# Autodesk Inventor assembly: MainAssy_MIR_MIR
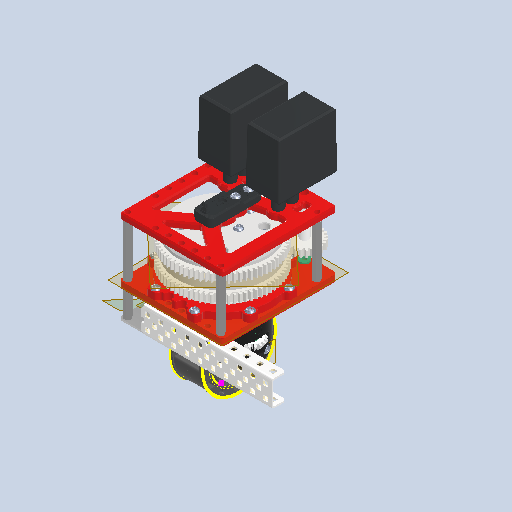
[picture p0: Inventor's stored thumbnail of the model, 512x512]
Saved by Autodesk Inventor 2023 (Build 270158000, 158)
## iProperties
Created: 2022-10-29
Part Number: MainAssy_MIR_MIR
Document SubType Name: Assembly
Designer: zac-h
Author: zac-h
## Documents named in this file (41)
- C:\Users\Zac Hah\Documents\GitHub\spin-up-cad\guardSwerve5\MainAssy_MIR_MIR.iam
- C:\Users\Zac Hah\Documents\GitHub\spin-up-cad\guardSwerve5\WheelHalf_MIR1_MIR.ipt
- C:\Users\Zac Hah\Documents\GitHub\spin-up-cad\guardSwerve5\WheelHalf_MIR_MIR_MIR.ipt
- C:\Users\Zac Hah\Documents\GitHub\spin-up-cad\guardSwerve5\Carriage_MIR_MIR.ipt
- C:\Users\Zac Hah\Documents\GitHub\spin-up-cad\guardSwerve5\MainAssy\Design Accelerator\Bevel Gears1_MIR_MIR.iam
- C:\Users\Zac Hah\Documents\GitHub\spin-up-cad\VEX-CAD-Inventor-1.3.0\VEX-CAD-Inventor-1.3.0\Motion\Circle Insert_MIR_MIR.ipt
- C:\Users\Zac Hah\Documents\GitHub\spin-up-cad\guardSwerve5\Baseplate_MIR_MIR.ipt
- C:\Users\Zac Hah\Documents\GitHub\spin-up-cad\VEX-CAD-Inventor-1.3.0\VEX-CAD-Inventor-1.3.0\Structure\C-Channels\Aluminum 1x2x1\Alu C 1x2x1x10_MIR_MIR.ipt
- C:\Users\Zac Hah\Documents\GitHub\spin-up-cad\guardSwerve5\UpperRaceRing_MIR_MIR.ipt
- C:\Users\Zac Hah\Documents\GitHub\spin-up-cad\guardSwerve5\SteeringCoupler_MIR_MIR.ipt
- C:\Users\Zac Hah\Documents\GitHub\spin-up-cad\guardSwerve5\MainAssy\Design Accelerator\Spur Gears1_MIR_MIR.iam
- C:\Users\Zac Hah\Documents\GitHub\spin-up-cad\guardSwerve5\MainAssy\Design Accelerator\Spur Gears2_MIR_MIR.iam
- C:\Users\Zac Hah\Documents\GitHub\spin-up-cad\guardSwerve5\MainAssy\Design Accelerator\Spur Gears4_MIR_MIR.iam
- C:\Users\Zac Hah\Documents\GitHub\spin-up-cad\guardSwerve5\MainAssy\Design Accelerator\Spur Gears5_MIR_MIR.iam
- C:\Users\Zac Hah\Documents\GitHub\spin-up-cad\guardSwerve5\MainAssy\Design Accelerator\Spur Gears3_MIR_MIR.iam
- C:\Users\Zac Hah\Documents\GitHub\spin-up-cad\guardSwerve5\MainAssy\Design Accelerator\Spur Gears6_MIR_MIR.iam
- C:\Users\Zac Hah\Documents\GitHub\spin-up-cad\guardSwerve5\UpperRingSeat_MIR_MIR.ipt
- C:\Users\Zac Hah\Documents\GitHub\spin-up-cad\VEX-CAD-Inventor-1.3.0\VEX-CAD-Inventor-1.3.0\Structure\Hardware\Screw Steel - Star\SScrew Star Smooth 1.000.ipt
- C:\Users\zac-h\Documents\CAD\VEX-CAD-Inventor-1.3.0\VEX-CAD-Inventor-1.3.0\Structure\Hardware\Screw Steel - Star.ipt
- C:\Users\Zac Hah\Documents\GitHub\spin-up-cad\guardSwerve5\DiffCap_MIR_MIR.ipt
- C:\Users\Zac Hah\Documents\GitHub\spin-up-cad\VEX-CAD-Inventor-1.3.0\VEX-CAD-Inventor-1.3.0\Motion\Square Insert_MIR_MIR.ipt
- C:\Users\Zac Hah\Documents\GitHub\spin-up-cad\VEX-CAD-Inventor-1.3.0\VEX-CAD-Inventor-1.3.0\Structure\Hardware\Screw Steel - Star\SScrew Star Smooth .875.ipt
- C:\Users\Zac Hah\Documents\GitHub\spin-up-cad\VEX-CAD-Inventor-1.3.0\VEX-CAD-Inventor-1.3.0\Structure\Hardware\Nut Nylock_MIR2_MIR.ipt
- C:\Users\Zac Hah\Documents\GitHub\spin-up-cad\VEX-CAD-Inventor-1.3.0\VEX-CAD-Inventor-1.3.0\Motion\Shaft LS\Shaft LS 3.0 in.ipt
- C:\Users\zac-h\Documents\CAD\VEX-CAD-Inventor-1.3.0\VEX-CAD-Inventor-1.3.0\Motion\Shaft LS.ipt
- C:\Users\Zac Hah\Documents\GitHub\spin-up-cad\VEX-CAD-Inventor-1.3.0\VEX-CAD-Inventor-1.3.0\Structure\Hardware\Screw Steel - Star\SScrew Star Smooth 1.750.ipt
- C:\Users\Zac Hah\Documents\GitHub\spin-up-cad\VEX-CAD-Inventor-1.3.0\VEX-CAD-Inventor-1.3.0\Structure\Standoff\Standoff 2.00.ipt
- C:\Users\zac-h\Documents\CAD\VEX-CAD-Inventor-1.3.0\VEX-CAD-Inventor-1.3.0\Structure\Standoff.ipt
- C:\Users\Zac Hah\Documents\GitHub\spin-up-cad\guardSwerve5\TopPlate_MIR_MIR.ipt
- C:\Users\Zac Hah\Documents\GitHub\spin-up-cad\VEX-CAD-Inventor-1.3.0\VEX-CAD-Inventor-1.3.0\Electronics\V5 Simple Motor_MIR2_MIR.ipt
- C:\Users\Zac Hah\Documents\GitHub\spin-up-cad\VEX-CAD-Inventor-1.3.0\VEX-CAD-Inventor-1.3.0\Electronics\Sensors\Potentiometer V2_MIR_MIR.ipt
- C:\Users\Zac Hah\Documents\GitHub\spin-up-cad\VEX-CAD-Inventor-1.3.0\VEX-CAD-Inventor-1.3.0\Structure\Hardware\Screw Steel - Star\SScrew Star Smooth .750.ipt
- C:\Users\Zac Hah\Documents\GitHub\spin-up-cad\VEX-CAD-Inventor-1.3.0\VEX-CAD-Inventor-1.3.0\Structure\Hardware\Screw Steel - Star\SScrew Star Smooth .500.ipt
- C:\Users\Zac Hah\Documents\GitHub\spin-up-cad\guardSwerve5\UnderGusset_MIR_MIR.ipt
- C:\Users\Zac Hah\Documents\GitHub\spin-up-cad\VEX-CAD-Inventor-1.3.0\VEX-CAD-Inventor-1.3.0\Structure\Standoff\Standoff 1.00.ipt
- C:\Users\Zac Hah\Documents\GitHub\spin-up-cad\guardSwerve5\1.2inSpacer_MIR_MIR.ipt
- C:\Users\Zac Hah\Documents\GitHub\spin-up-cad\guardSwerve1\bearingsleeve_MIR2_MIR.ipt
- C:\Users\Zac Hah\Documents\GitHub\spin-up-cad\guardSwerve5\608bearing_MIR_MIR.ipt
- C:\Users\Zac Hah\Documents\GitHub\spin-up-cad\VEX-CAD-Inventor-1.3.0\VEX-CAD-Inventor-1.3.0\Structure\Hardware\Screw Steel - Star\SScrew Star Smooth .250.ipt
- C:\Users\Zac Hah\Documents\GitHub\spin-up-cad\VEX-CAD-Inventor-1.3.0\VEX-CAD-Inventor-1.3.0\Structure\Hardware\Screw Steel - Star\SScrew Star Smooth 1.250.ipt
- C:\Users\Zac Hah\Documents\GitHub\spin-up-cad\VEX-CAD-Inventor-1.3.0\VEX-CAD-Inventor-1.3.0\Motion\0.188 ID x 0.500 OD x 0.196 WD (Radial Bearing) (217-3246).step
## Components (84 placed, 36 different names)
1. WheelHalf_MIR1_MIR:1 — Mate:1
2. WheelHalf_MIR_MIR_MIR:1 — Flush:1, Mate:25, Angle:5
3. Carriage_MIR_MIR:1 — Flush:1, Mate:4, Mate:24, Angle:4, Mate:5, Mate:6, Mate:7, Insert:11, Insert:12, Flush:2, Insert:3, Insert:39, Insert:38, Insert:37, Insert:36
4. Bevel Gears1_MIR_MIR:1 [sub-assembly] — Mate:1, Mate:4, Mate:24, Angle:4, Mate:25, Angle:5
5. Circle Insert_MIR_MIR:1 — Mate:5, Mate:6, Mate:7
6. Circle Insert_MIR_MIR:2 — Insert:49
7. Circle Insert_MIR_MIR:3 — Insert:44
8. Baseplate_MIR_MIR:1 — Flush:2, Insert:14, Insert:21, Insert:15, Insert:16, Flush:3, Flush:4, Insert:28, Insert:27, Insert:69, Insert:66, Insert:67, Insert:68
9. Alu C 1x2x1x10_MIR_MIR:1 — Insert:14, Insert:21, Flush:13, Flush:14
10. Alu C 1x2x1x10_MIR_MIR:2 — Insert:15, Insert:16
11. UpperRaceRing_MIR_MIR:1 — Flush:3, Flush:4, Insert:29
12. SteeringCoupler_MIR_MIR:1 — Flush:5, Insert:31, Mate:20, Mate:21, Insert:32, Insert:33, Insert:34, Flush:8, Insert:45, Insert:63, Insert:64, Insert:65
13. Spur Gears1_MIR_MIR:1 [sub-assembly] — Insert:31, Insert:49, Flush:7
14. Spur Gears2_MIR_MIR:1 [sub-assembly] — Mate:20, Mate:21, Insert:30, Mate:23, Flush:11
15. Spur Gears4_MIR_MIR:1 [sub-assembly] — Insert:30, Mate:23, Flush:11
16. Circle Insert_MIR_MIR:4 — Insert:28, Insert:85
17. Circle Insert_MIR_MIR:5 — Insert:27, Mate:15
18. Spur Gears5_MIR_MIR:1 [sub-assembly] — Mate:15, Flush:7, Flush:15
19. Spur Gears3_MIR_MIR:1 [sub-assembly] — Insert:32, Insert:43
20. Spur Gears3_MIR_MIR:2 [sub-assembly] — Insert:33, Insert:44
21. Spur Gears6_MIR_MIR:1 [sub-assembly] — Insert:34, Insert:42
22. UpperRingSeat_MIR_MIR:1 — Flush:8, Insert:35, Flush:9, Flush:10, Insert:48
23. Spur Gears1_MIR_MIR:2 [sub-assembly] — Insert:35, Insert:51
24. SScrew Star Smooth 1.000:1 — Insert:39
25. SScrew Star Smooth 1.000:2 — Insert:38
26. SScrew Star Smooth 1.000:3 — Insert:37
27. SScrew Star Smooth 1.000:4 — Insert:36
28. Spur Gears4_MIR_MIR:2 [sub-assembly]
29. DiffCap_MIR_MIR:1 — Flush:9, Flush:10, Insert:62, Insert:61, Insert:60
30. Square Insert_MIR_MIR:1 — Insert:42
31. Circle Insert_MIR_MIR:6 — Insert:43
32. SScrew Star Smooth .875:5 — Insert:45
33. Nut Nylock_MIR2_MIR:1 — Insert:48
34. Circle Insert_MIR_MIR:7 — Insert:51
35. Shaft LS 3.0 in:1
36. SScrew Star Smooth 1.750:6 — Insert:62
37. SScrew Star Smooth 1.750:7 — Insert:61
38. SScrew Star Smooth 1.750:8 — Insert:60
39. Nut Nylock_MIR2_MIR:2 — Insert:63
40. Nut Nylock_MIR2_MIR:3 — Insert:64
41. Nut Nylock_MIR2_MIR:4 — Insert:65
42. Standoff 2.00:1 — Insert:69
43. Standoff 2.00:2 — Insert:66
44. Standoff 2.00:3 — Insert:67
45. Standoff 2.00:4 — Insert:68, Flush:12
46. TopPlate_MIR_MIR:1 — Flush:12, Insert:72, Insert:73, Insert:70, Insert:71, Insert:80, Insert:77, Insert:78, Insert:79
47. V5 Simple Motor_MIR2_MIR:1 — Insert:72, Insert:73
48. V5 Simple Motor_MIR2_MIR:2 — Insert:70, Insert:71
49. Potentiometer V2_MIR_MIR:1 — Insert:80, Insert:81, Insert:82
50. SScrew Star Smooth .750:9
51. SScrew Star Smooth .750:10 — Insert:77
52. SScrew Star Smooth .750:11 — Insert:78
53. SScrew Star Smooth .750:12 — Insert:79
54. SScrew Star Smooth .500:13 — Insert:81
55. SScrew Star Smooth .500:14 — Insert:82
56. UnderGusset_MIR_MIR:1 — Flush:13, Flush:14, Insert:83, Insert:84
57. Standoff 1.00:5 — Insert:83
58. SScrew Star Smooth .500:15 — Insert:84
59. 1.2inSpacer_MIR_MIR:1 — Flush:15
60. Spur Gears5_MIR_MIR:2 [sub-assembly] — Insert:85
61. SScrew Star Smooth .250:16 — Insert:11
62. SScrew Star Smooth .250:17 — Insert:12
63. SScrew Star Smooth .250:20
64. SScrew Star Smooth .250:21
65. bearingsleeve_MIR2_MIR:1 — Insert:3, Insert:2
66. 608bearing_MIR_MIR:1 — Insert:2, Flush:5
67. bearingsleeve_MIR2_MIR:2
68. 608bearing_MIR_MIR:2
69. bearingsleeve_MIR2_MIR:3
70. 608bearing_MIR_MIR:3
71. bearingsleeve_MIR2_MIR:4
72. 608bearing_MIR_MIR:4
73. SScrew Star Smooth .500:18 — Insert:29
74. SScrew Star Smooth .500:22
75. SScrew Star Smooth .500:23
76. SScrew Star Smooth .500:24
77. SScrew Star Smooth .500:25
78. SScrew Star Smooth .500:26
79. SScrew Star Smooth .500:27
80. SScrew Star Smooth .500:28
81. SScrew Star Smooth 1.250:19
82. SScrew Star Smooth 1.250:29
83. SScrew Star Smooth 1.250:30
84. SScrew Star Smooth 1.250:31
## Component patterns: (2 elements, first: SScrew Star Smooth .250:16 + SScrew Star Smooth .250:17), (4 elements, first: bearingsleeve_MIR2_MIR:1 + 608bearing_MIR_MIR:1), (8 elements, first: SScrew Star Smooth .500:18), (4 elements, first: SScrew Star Smooth 1.250:19)
## Relationships (78: Insert 51, Flush 14, Mate 11, Angle 2)
- Flush:1: WheelHalf_MIR_MIR_MIR:1 ↔ Carriage_MIR_MIR:1
- Mate:1: WheelHalf_MIR1_MIR:1 ↔ Bevel Gears1_MIR_MIR:1
- Mate:4: Carriage_MIR_MIR:1 ↔ Bevel Gears1_MIR_MIR:1
- Mate:24: Carriage_MIR_MIR:1 ↔ Bevel Gears1_MIR_MIR:1
- Angle:4 (0 deg): Carriage_MIR_MIR:1 ↔ Bevel Gears1_MIR_MIR:1
- Mate:25: WheelHalf_MIR_MIR_MIR:1 ↔ Bevel Gears1_MIR_MIR:1
- Angle:5 (0 deg): WheelHalf_MIR_MIR_MIR:1 ↔ Bevel Gears1_MIR_MIR:1
- Mate:5: Carriage_MIR_MIR:1 ↔ Circle Insert_MIR_MIR:1
- Mate:6: Carriage_MIR_MIR:1 ↔ Circle Insert_MIR_MIR:1
- Mate:7: Carriage_MIR_MIR:1 ↔ Circle Insert_MIR_MIR:1
- Insert:11: Carriage_MIR_MIR:1 ↔ SScrew Star Smooth .250:16
- Insert:12: Carriage_MIR_MIR:1 ↔ SScrew Star Smooth .250:17
- Flush:2: Carriage_MIR_MIR:1 ↔ Baseplate_MIR_MIR:1
- Insert:14: Baseplate_MIR_MIR:1 ↔ Alu C 1x2x1x10_MIR_MIR:1
- Insert:21: Baseplate_MIR_MIR:1 ↔ Alu C 1x2x1x10_MIR_MIR:1
- Insert:15: Baseplate_MIR_MIR:1 ↔ Alu C 1x2x1x10_MIR_MIR:2
- Insert:16: Baseplate_MIR_MIR:1 ↔ Alu C 1x2x1x10_MIR_MIR:2
- Flush:3: Baseplate_MIR_MIR:1 ↔ UpperRaceRing_MIR_MIR:1
- Flush:4: Baseplate_MIR_MIR:1 ↔ UpperRaceRing_MIR_MIR:1
- Insert:3: Carriage_MIR_MIR:1 ↔ bearingsleeve_MIR2_MIR:1
- Insert:2: bearingsleeve_MIR2_MIR:1 ↔ 608bearing_MIR_MIR:1
- Flush:5: SteeringCoupler_MIR_MIR:1 ↔ 608bearing_MIR_MIR:1
- Insert:31: SteeringCoupler_MIR_MIR:1 ↔ Spur Gears1_MIR_MIR:1
- Insert:49: Circle Insert_MIR_MIR:2 ↔ Spur Gears1_MIR_MIR:1
- Mate:20: SteeringCoupler_MIR_MIR:1 ↔ Spur Gears2_MIR_MIR:1
- Mate:21: SteeringCoupler_MIR_MIR:1 ↔ Spur Gears2_MIR_MIR:1
- Insert:30: Spur Gears2_MIR_MIR:1 ↔ Spur Gears4_MIR_MIR:1
- Mate:23: Spur Gears2_MIR_MIR:1 ↔ Spur Gears4_MIR_MIR:1
- Flush:11: Spur Gears2_MIR_MIR:1 ↔ Spur Gears4_MIR_MIR:1
- Insert:28: Baseplate_MIR_MIR:1 ↔ Circle Insert_MIR_MIR:4
- Insert:27: Baseplate_MIR_MIR:1 ↔ Circle Insert_MIR_MIR:5
- Mate:15: Circle Insert_MIR_MIR:5 ↔ Spur Gears5_MIR_MIR:1
- Flush:7: Spur Gears1_MIR_MIR:1 ↔ Spur Gears5_MIR_MIR:1
- Insert:29: UpperRaceRing_MIR_MIR:1 ↔ SScrew Star Smooth .500:18
- Insert:32: SteeringCoupler_MIR_MIR:1 ↔ Spur Gears3_MIR_MIR:1
- Insert:33: SteeringCoupler_MIR_MIR:1 ↔ Spur Gears3_MIR_MIR:2
- Insert:44: Circle Insert_MIR_MIR:3 ↔ Spur Gears3_MIR_MIR:2
- Insert:34 (1.27 mm): SteeringCoupler_MIR_MIR:1 ↔ Spur Gears6_MIR_MIR:1
- Flush:8: SteeringCoupler_MIR_MIR:1 ↔ UpperRingSeat_MIR_MIR:1
- Insert:35: UpperRingSeat_MIR_MIR:1 ↔ Spur Gears1_MIR_MIR:2
- Insert:39: Carriage_MIR_MIR:1 ↔ SScrew Star Smooth 1.000:1
- Insert:38: Carriage_MIR_MIR:1 ↔ SScrew Star Smooth 1.000:2
- Insert:37: Carriage_MIR_MIR:1 ↔ SScrew Star Smooth 1.000:3
- Insert:36: Carriage_MIR_MIR:1 ↔ SScrew Star Smooth 1.000:4
- Flush:9: UpperRingSeat_MIR_MIR:1 ↔ DiffCap_MIR_MIR:1
- Flush:10: UpperRingSeat_MIR_MIR:1 ↔ DiffCap_MIR_MIR:1
- Insert:42: Spur Gears6_MIR_MIR:1 ↔ Square Insert_MIR_MIR:1
- Insert:43: Spur Gears3_MIR_MIR:1 ↔ Circle Insert_MIR_MIR:6
- Insert:45: SteeringCoupler_MIR_MIR:1 ↔ SScrew Star Smooth .875:5
- Insert:48: UpperRingSeat_MIR_MIR:1 ↔ Nut Nylock_MIR2_MIR:1
- Insert:51: Spur Gears1_MIR_MIR:2 ↔ Circle Insert_MIR_MIR:7
- Insert:62: DiffCap_MIR_MIR:1 ↔ SScrew Star Smooth 1.750:6
- Insert:61: DiffCap_MIR_MIR:1 ↔ SScrew Star Smooth 1.750:7
- Insert:60: DiffCap_MIR_MIR:1 ↔ SScrew Star Smooth 1.750:8
- Insert:63: SteeringCoupler_MIR_MIR:1 ↔ Nut Nylock_MIR2_MIR:2
- Insert:64: SteeringCoupler_MIR_MIR:1 ↔ Nut Nylock_MIR2_MIR:3
- Insert:65: SteeringCoupler_MIR_MIR:1 ↔ Nut Nylock_MIR2_MIR:4
- Insert:69: Baseplate_MIR_MIR:1 ↔ Standoff 2.00:1
- Insert:66: Baseplate_MIR_MIR:1 ↔ Standoff 2.00:2
- Insert:67: Baseplate_MIR_MIR:1 ↔ Standoff 2.00:3
- Insert:68: Baseplate_MIR_MIR:1 ↔ Standoff 2.00:4
- Flush:12: Standoff 2.00:4 ↔ TopPlate_MIR_MIR:1
- Insert:72: TopPlate_MIR_MIR:1 ↔ V5 Simple Motor_MIR2_MIR:1
- Insert:73: TopPlate_MIR_MIR:1 ↔ V5 Simple Motor_MIR2_MIR:1
- Insert:70: TopPlate_MIR_MIR:1 ↔ V5 Simple Motor_MIR2_MIR:2
- Insert:71: TopPlate_MIR_MIR:1 ↔ V5 Simple Motor_MIR2_MIR:2
- Insert:80: TopPlate_MIR_MIR:1 ↔ Potentiometer V2_MIR_MIR:1
- Insert:77: TopPlate_MIR_MIR:1 ↔ SScrew Star Smooth .750:10
- Insert:78: TopPlate_MIR_MIR:1 ↔ SScrew Star Smooth .750:11
- Insert:79: TopPlate_MIR_MIR:1 ↔ SScrew Star Smooth .750:12
- Insert:81: Potentiometer V2_MIR_MIR:1 ↔ SScrew Star Smooth .500:13
- Insert:82: Potentiometer V2_MIR_MIR:1 ↔ SScrew Star Smooth .500:14
- Flush:13: Alu C 1x2x1x10_MIR_MIR:1 ↔ UnderGusset_MIR_MIR:1
- Flush:14: Alu C 1x2x1x10_MIR_MIR:1 ↔ UnderGusset_MIR_MIR:1
- Insert:83: UnderGusset_MIR_MIR:1 ↔ Standoff 1.00:5
- Insert:84: UnderGusset_MIR_MIR:1 ↔ SScrew Star Smooth .500:15
- Flush:15: Spur Gears5_MIR_MIR:1 ↔ 1.2inSpacer_MIR_MIR:1
- Insert:85 (28.575 mm): Circle Insert_MIR_MIR:4 ↔ Spur Gears5_MIR_MIR:2
